# Autodesk Inventor assembly: Piston Wall Guide Small assy
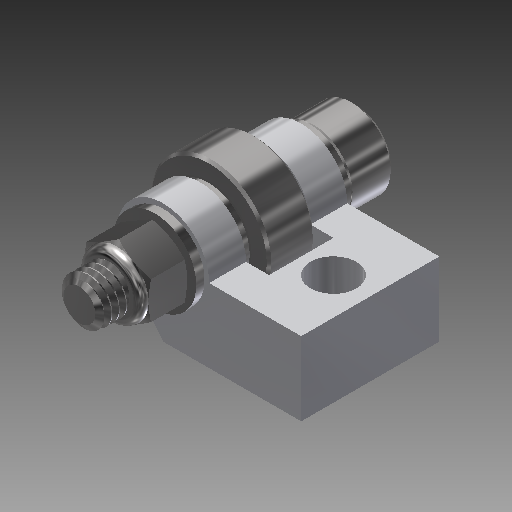
[picture p0: Inventor's stored thumbnail of the model, 512x512]
Saved by Autodesk Inventor 2018 (Build 220112000, 112)
## iProperties
Created: 2017-09-27
Part Number: Piston Wall Guide Small assy
Document SubType Name: Assembly
Designer: Gabriel Smolnycki
Author: Gabriel Smolnycki
## Documents named in this file (6)
- E:\planb\mechanics\Subassemblies\Piston Wall Guide Small assy.iam
- E:\planb\mechanics\Piston\Piston Wall Guide Small.ipt
- E:\planb\mechanics\Hardware\M4 SS Washer.ipt
- E:\planb\mechanics\Hardware\4x13 SS Ball Bearing (7804K103).ipt
- E:\planb\mechanics\Hardware\M4 SS Locknut.ipt
- E:\planb\mechanics\Hardware\M4x25 SS SHCS.ipt
## Components (8 placed, 5 different names)
1. Piston Wall Guide Small:1 — Insert:1, Mate:1, Insert:3, Insert:4, Insert:5
2. M4 SS Washer:1 — Insert:1, Insert:2
3. M4 SS Washer:2 — Insert:3
4. M4 SS Washer:3 — Insert:4, Insert:6
5. M4 SS Washer:4 — Insert:5, Insert:7
6. 4x13 SS Ball Bearing (7804K103):1 — Mate:1, Insert:2
7. M4 SS Locknut:1 — Insert:7
8. M4x25 SS SHCS:1 — Insert:6
## Relationships (8: Insert 7, Mate 1)
- Insert:1: Piston Wall Guide Small:1 ↔ M4 SS Washer:1
- Mate:1: Piston Wall Guide Small:1 ↔ 4x13 SS Ball Bearing (7804K103):1
- Insert:2: M4 SS Washer:1 ↔ 4x13 SS Ball Bearing (7804K103):1
- Insert:3: Piston Wall Guide Small:1 ↔ M4 SS Washer:2
- Insert:4: Piston Wall Guide Small:1 ↔ M4 SS Washer:3
- Insert:5: Piston Wall Guide Small:1 ↔ M4 SS Washer:4
- Insert:6: M4 SS Washer:3 ↔ M4x25 SS SHCS:1
- Insert:7: M4 SS Washer:4 ↔ M4 SS Locknut:1
